# Autodesk Inventor assembly: DStation
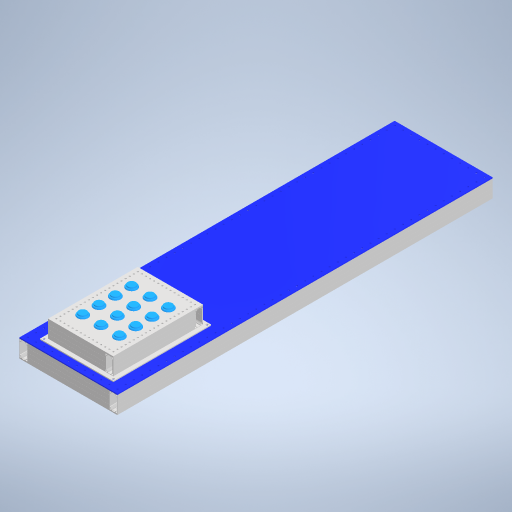
[picture p0: Inventor's stored thumbnail of the model, 512x512]
Saved by Autodesk Inventor 2023.4 (Build 274418000, 418)
## iProperties
Created: 2023-12-21
Part Number: DStation
Document SubType Name: Assembly
Designer: elija
Author: elija
## Documents named in this file (6)
- C:\Users\amrom\OneDrive\Documents\GIT Hub\2024-CAD\Driver's station\DStation.iam
- C:\Users\amrom\OneDrive\Documents\GIT Hub\2024-CAD\Driver's station\REV MAXTUBE 10.ipt
- C:\Users\amrom\OneDrive\Documents\GIT Hub\2024-CAD\Driver's station\REV 46 MAXTUBE.ipt
- C:\Users\amrom\OneDrive\Documents\GIT Hub\2024-CAD\Driver's station\TOP DS new.ipt
- C:\Users\amrom\OneDrive\Documents\GIT Hub\2024-CAD\Driver's station\BOTTOM DS new.ipt
- C:\Users\amrom\OneDrive\Documents\GIT Hub\2024-CAD\Driver's station\Button Box\Button Box Assembly.iam
## Components (7 placed, 5 different names)
1. REV MAXTUBE 10:1 — Flush:11, Flush:13
2. REV MAXTUBE 10:2 — Mate:42
3. REV 46 MAXTUBE:1
4. REV 46 MAXTUBE:2 — Flush:10, Mate:43, Flush:12
5. TOP DS new:1 — Mate:42, Flush:10, Flush:11, Mate:45, Mate:46
6. BOTTOM DS new:1 — Mate:43, Flush:12, Flush:13, Mate:44
7. Button Box Assembly:1 [sub-assembly] — Mate:44, Mate:45, Mate:46
## Relationships (9: Mate 5, Flush 4)
- Mate:42: REV MAXTUBE 10:2 ↔ TOP DS new:1
- Flush:10: REV 46 MAXTUBE:2 ↔ TOP DS new:1
- Flush:11: REV MAXTUBE 10:1 ↔ TOP DS new:1
- Mate:43: REV 46 MAXTUBE:2 ↔ BOTTOM DS new:1
- Flush:12: REV 46 MAXTUBE:2 ↔ BOTTOM DS new:1
- Flush:13: REV MAXTUBE 10:1 ↔ BOTTOM DS new:1
- Mate:44: BOTTOM DS new:1 ↔ Button Box Assembly:1
- Mate:45: TOP DS new:1 ↔ Button Box Assembly:1
- Mate:46: TOP DS new:1 ↔ Button Box Assembly:1
